# Autodesk Inventor assembly: mg996r 3mm right leg
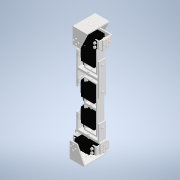
[picture p0: Inventor's stored thumbnail of the model, 180x180]
Saved by Autodesk Inventor 2021.4 (Build 254397000, 397)
## iProperties
Created: 2022-07-09
Part Number: mg996r 3mm right leg
Document SubType Name: Assembly
Designer: isamu
Author: isamu
## Documents named in this file (5)
- D:\personal_projects\robot\inventor\2021\mg996r 3mm right leg.iam
- D:\personal_projects\robot\inventor\2021\mg996r 3mm frame middle leg.iam
- D:\personal_projects\robot\inventor\2021\base mg996r 3mm centered right.iam
- D:\personal_projects\robot\inventor\2021\base mg996r 3mm right foot.iam
- D:\personal_projects\robot\exports\screws\m3 nuts.ipt
## Components (13 placed, 4 different names)
1. mg996r 3mm frame middle leg:1 [sub-assembly] — Mate:1, Mate:2, Mate:3, Mate:4, Mate:5, Mate:6
2. base mg996r 3mm centered right:1 [sub-assembly] — Mate:1, Mate:2, Mate:3, Insert:1, Insert:2, Insert:3, Insert:4, Insert:5
3. base mg996r 3mm right foot:1 [sub-assembly] — Mate:4, Mate:5, Mate:6, Insert:6, Insert:7, Insert:8, Insert:9, Insert:10
4. m3 nuts:1 — Insert:8
5. m3 nuts:2 — Insert:6
6. m3 nuts:3 — Insert:10
7. m3 nuts:4 — Insert:9
8. m3 nuts:5 — Insert:7
9. m3 nuts:6 — Insert:1
10. m3 nuts:7 — Insert:5
11. m3 nuts:8 — Insert:4
12. m3 nuts:9 — Insert:3
13. m3 nuts:10 — Insert:2
## Relationships (16: Insert 10, Mate 6)
- Mate:1: mg996r 3mm frame middle leg:1 ↔ base mg996r 3mm centered right:1
- Mate:2: mg996r 3mm frame middle leg:1 ↔ base mg996r 3mm centered right:1
- Mate:3: mg996r 3mm frame middle leg:1 ↔ base mg996r 3mm centered right:1
- Insert:1: base mg996r 3mm centered right:1 ↔ m3 nuts:6
- Insert:2: base mg996r 3mm centered right:1 ↔ m3 nuts:10
- Insert:3: base mg996r 3mm centered right:1 ↔ m3 nuts:9
- Insert:4: base mg996r 3mm centered right:1 ↔ m3 nuts:8
- Insert:5: base mg996r 3mm centered right:1 ↔ m3 nuts:7
- Mate:4: mg996r 3mm frame middle leg:1 ↔ base mg996r 3mm right foot:1
- Mate:5: mg996r 3mm frame middle leg:1 ↔ base mg996r 3mm right foot:1
- Mate:6: mg996r 3mm frame middle leg:1 ↔ base mg996r 3mm right foot:1
- Insert:6: base mg996r 3mm right foot:1 ↔ m3 nuts:2
- Insert:7: base mg996r 3mm right foot:1 ↔ m3 nuts:5
- Insert:8: base mg996r 3mm right foot:1 ↔ m3 nuts:1
- Insert:9: base mg996r 3mm right foot:1 ↔ m3 nuts:4
- Insert:10: base mg996r 3mm right foot:1 ↔ m3 nuts:3
